# Autodesk Inventor assembly: LR_03
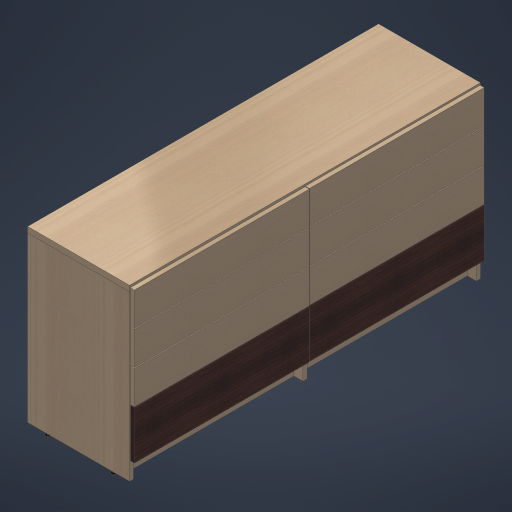
[picture p0: Inventor's stored thumbnail of the model, 512x512]
Saved by Autodesk Inventor 2024.3 (Build 283343000, 343)
## iProperties
Created: 2013-04-03
Part Number: LR_03
Document SubType Name: Assembly
Designer: User
Description: Commode
Material Code: Item.FillWorkpiece.Material.Code
Author: User
## Documents named in this file (21)
- C:\W4INV 2024 Design\PROJECTS\Living Room\Commode\LR_03.iam
- C:\W4INV 2024 Design\PROJECTS\Samples\Living Room\Commode\LR_0309.ipt
- C:\W4INV 2024 Design\PROJECTS\Samples\Living Room\Commode\LR_0304.ipt
- C:\W4INV 2024 Design\PROJECTS\Samples\Living Room\Commode\LR_0301.ipt
- C:\W4INV 2024 Design\PROJECTS\Samples\Living Room\Commode\LR_0308.ipt
- C:\W4INV 2024 Design\PROJECTS\Samples\Living Room\Commode\LR_0306.ipt
- C:\W4INV 2024 Design\PROJECTS\Samples\Living Room\Commode\LR_0303.ipt
- C:\W4INV 2024 Design\PROJECTS\Samples\Living Room\Commode\LR_0307.ipt
- C:\W4INV 2024 Design\PROJECTS\Samples\Living Room\Commode\LR_0302.ipt
- C:\W4INV 2024 Design\PROJECTS\Samples\Living Room\Commode\LR_0305.ipt
- C:\W4INV 2024 Design\PROJECTS\Samples\Living Room\Commode\SkeletonLR_030000.ipt
- C:\W4INV 2024 Design\PROJECTS\Samples\Living Room\Commode\LR_0300.ipt
- C:\W4INV 2024 Design\PROJECTS\Samples\Living Room\Commode\LR_0310.ipt
- C:\W4INV 2024 Design\PROJECTS\Samples\Living Room\Commode\LR_03\iCopy\iCopy1\LR_0311Full Pull Drawer1.iam
- C:\W4INV 2024 Design\PROJECTS\Samples\Living Room\Commode\LR_03\iCopy\iCopy2\LR_0312Full Pull Drawer1.iam
- C:\W4INV 2024 Design\_LIBRARY\Fixed joints\Minifix joint\MINIFIX D15 v2\Minifix D15 & Dowel L34 & Cap D15 PB T18 LH.ipt
- C:\W4INV 2024 Design\_LIBRARY\Fixed joints\Minifix joint\MINIFIX D15 v2\Minifix D15 & Dowel L34 & Cap D15 PB T18 RH.ipt
- C:\W4INV 2024 Design\_LIBRARY\Supports and legs\Supports\ADJUSTABLE SUPPORT\Support M6 H27 D18 with Bushing SB T18.ipt
- C:\W4INV 2024 Design\LIBRARY\Supports and legs\Supports\ADJUSTABLE SUPPORT.ipt
- C:\W4INV 2024 Design\LIBRARY\Fixed joints\Minifix joint\MINIFIX D15 v2.ipt
- C:\W4INV 2023 Design\PROJECTS\Samples\Living Room\Commode\LR_03.iam
## Components (46 placed, 17 different names)
1. K Virsus::1 — Mate:107, Mate:109, Mate:111, Mate:113, Mate:115, Mate:117
2. K Kaire::1 — Flush:4, Flush:5, Mate:55, Mate:56, Mate:57, Mate:58, Mate:59, Mate:60, Mate:63, Flush:39, Flush:69, Mate:79, Mate:81, Mate:83, Flush:72, Mate:85, Mate:87, Mate:89, Mate:91, Mate:99, Flush:83, Flush:86
3. K Desine::1 — Flush:35, Flush:71, Flush:74, Mate:97, Mate:105, Flush:85, Flush:88
4. K Vertikali pertvara::1 — Mate:61, Mate:62, Flush:37, Flush:70, Flush:73, Mate:93, Mate:95, Mate:101, Mate:103, Flush:84, Flush:87
5. K Kairys dugnas::1 — Flush:75, Flush:76, Flush:77, Flush:78, Flush:79, Flush:80, Flush:81, Flush:82
6. K Desinys dugnas::1
7. K Desine nugarele::1
8. K Kaire nugarele::1
9. K Apatinis fasadas::1 — Flush:30, Mate:54
10. K Apatinis fasadas::2 — Flush:30, Mate:54, Flush:34
11. LR_0311Full Pull Drawer1:3 [sub-assembly] — Mate:61, Flush:35, Flush:36
12. Support M6 H27 D18 with Bushing SB T18:7 — Mate:78, Flush:69, Mate:79
13. Support M6 H27 D18 with Bushing SB T18:8 — Mate:80, Flush:70, Mate:81
14. Support M6 H27 D18 with Bushing SB T18:9 — Mate:82, Flush:71, Mate:83
15. Support M6 H27 D18 with Bushing SB T18:10 — Mate:84, Flush:72, Mate:85
16. Support M6 H27 D18 with Bushing SB T18:11 — Mate:86, Flush:73, Mate:87
17. Support M6 H27 D18 with Bushing SB T18:12 — Mate:88, Flush:74, Mate:89
18. Minifix D15 & Dowel L34 & Cap D15 PB T18 LH:1 — Mate:90, Mate:91, Flush:75
19. Minifix D15 & Dowel L34 & Cap D15 PB T18 LH:2 — Mate:92, Mate:93, Flush:76
20. Minifix D15 & Dowel L34 & Cap D15 PB T18 RH:3 — Mate:94, Mate:95, Flush:77
21. Minifix D15 & Dowel L34 & Cap D15 PB T18 LH:4 — Mate:96, Mate:97, Flush:78
22. Minifix D15 & Dowel L34 & Cap D15 PB T18 LH:5 — Mate:98, Mate:99, Flush:79
23. Minifix D15 & Dowel L34 & Cap D15 PB T18 RH:6 — Mate:100, Mate:101, Flush:80
24. Minifix D15 & Dowel L34 & Cap D15 PB T18 LH:7 — Mate:102, Mate:103, Flush:81
25. Minifix D15 & Dowel L34 & Cap D15 PB T18 RH:8 — Mate:104, Mate:105, Flush:82
26. Minifix D15 & Dowel L34 & Cap D15 PB T18 LH:9 — Mate:106, Flush:83, Mate:107
27. Minifix D15 & Dowel L34 & Cap D15 PB T18 RH:10 — Mate:108, Flush:84, Mate:109
28. Minifix D15 & Dowel L34 & Cap D15 PB T18 RH:11 — Mate:110, Flush:85, Mate:111
29. Minifix D15 & Dowel L34 & Cap D15 PB T18 RH:12 — Mate:112, Flush:86, Mate:113
30. Minifix D15 & Dowel L34 & Cap D15 PB T18 LH:13 — Mate:114, Flush:87, Mate:115
31. Minifix D15 & Dowel L34 & Cap D15 PB T18 LH:14 — Mate:116, Flush:88, Mate:117
32. LR_0311Full Pull Drawer1:1 [sub-assembly] — Mate:55, Mate:56, Mate:57, Flush:36
33. LR_0312Full Pull Drawer1:1 [sub-assembly] — Mate:58, Mate:59, Mate:60, Flush:38
34. K Plintusas::1
35. K Plintusas::2
36. LR_0312Full Pull Drawer1:2 [sub-assembly] — Mate:62, Flush:37, Flush:38
37. LR_0312Full Pull Drawer1:3 [sub-assembly] — Flush:40
38. LR_0312Full Pull Drawer1:4 [sub-assembly]
39. LR_0312Full Pull Drawer1:5 [sub-assembly] — Mate:63, Flush:39, Flush:40
40. LR_0312Full Pull Drawer1:6 [sub-assembly]
41. K Virsutinis fasadas::1 — Flush:33
42. K Virsutinis fasadas::2 — Flush:33, Flush:34
43. LR_0310:3
44. LR_0310:4
45. LR_0310:5
46. LR_0310:6
## Component patterns: (2 elements, first: K Plintusas::1), (3 elements, first: LR_0312Full Pull Drawer1:2), (2 elements, first: LR_0312Full Pull Drawer1:5), (3 elements, first: K Virsutinis fasadas::1 + K Virsutinis fasadas::2)
## Relationships (83: Mate 50, Flush 33)
- Flush:4 (-80 mm): K Kaire::1
- Flush:5 (-80 mm): K Kaire::1
- Flush:12 (-16 mm)
- Flush:13 (-16 mm)
- Flush:30: K Apatinis fasadas::1 ↔ K Apatinis fasadas::2
- Mate:54 (3 mm): K Apatinis fasadas::1 ↔ K Apatinis fasadas::2
- Flush:33: K Virsutinis fasadas::1 ↔ K Virsutinis fasadas::2
- Flush:34: K Apatinis fasadas::2 ↔ K Virsutinis fasadas::2
- Mate:55: K Kaire::1 ↔ LR_0311Full Pull Drawer1:1
- Mate:56: K Kaire::1 ↔ LR_0311Full Pull Drawer1:1
- Mate:57: K Kaire::1 ↔ LR_0311Full Pull Drawer1:1
- Mate:58: K Kaire::1 ↔ LR_0312Full Pull Drawer1:1
- Mate:59: K Kaire::1 ↔ LR_0312Full Pull Drawer1:1
- Mate:60: K Kaire::1 ↔ LR_0312Full Pull Drawer1:1
- Mate:61: K Vertikali pertvara::1 ↔ LR_0311Full Pull Drawer1:3
- Flush:35: K Desine::1 ↔ LR_0311Full Pull Drawer1:3
- Flush:36: LR_0311Full Pull Drawer1:3 ↔ LR_0311Full Pull Drawer1:1
- Mate:62: K Vertikali pertvara::1 ↔ LR_0312Full Pull Drawer1:2
- Flush:37: K Vertikali pertvara::1 ↔ LR_0312Full Pull Drawer1:2
- Flush:38: LR_0312Full Pull Drawer1:1 ↔ LR_0312Full Pull Drawer1:2
- Mate:63: K Kaire::1 ↔ LR_0312Full Pull Drawer1:5
- Flush:39: K Kaire::1 ↔ LR_0312Full Pull Drawer1:5
- Flush:40: LR_0312Full Pull Drawer1:3 ↔ LR_0312Full Pull Drawer1:5
- Mate:78: Support M6 H27 D18 with Bushing SB T18:7
- Flush:69 (9 mm): K Kaire::1 ↔ Support M6 H27 D18 with Bushing SB T18:7
- Mate:79 (17.5 mm): K Kaire::1 ↔ Support M6 H27 D18 with Bushing SB T18:7
- Mate:80: Support M6 H27 D18 with Bushing SB T18:8
- Flush:70 (9 mm): K Vertikali pertvara::1 ↔ Support M6 H27 D18 with Bushing SB T18:8
- Mate:81 (17.5 mm): K Kaire::1 ↔ Support M6 H27 D18 with Bushing SB T18:8
- Mate:82: Support M6 H27 D18 with Bushing SB T18:9
- Flush:71 (9 mm): K Desine::1 ↔ Support M6 H27 D18 with Bushing SB T18:9
- Mate:83 (17.5 mm): K Kaire::1 ↔ Support M6 H27 D18 with Bushing SB T18:9
- Mate:84: Support M6 H27 D18 with Bushing SB T18:10
- Flush:72 (9 mm): K Kaire::1 ↔ Support M6 H27 D18 with Bushing SB T18:10
- Mate:85 (17.5 mm): K Kaire::1 ↔ Support M6 H27 D18 with Bushing SB T18:10
- Mate:86: Support M6 H27 D18 with Bushing SB T18:11
- Flush:73 (9 mm): K Vertikali pertvara::1 ↔ Support M6 H27 D18 with Bushing SB T18:11
- Mate:87 (17.5 mm): K Kaire::1 ↔ Support M6 H27 D18 with Bushing SB T18:11
- Mate:88: Support M6 H27 D18 with Bushing SB T18:12
- Flush:74 (9 mm): K Desine::1 ↔ Support M6 H27 D18 with Bushing SB T18:12
- Mate:89 (17.5 mm): K Kaire::1 ↔ Support M6 H27 D18 with Bushing SB T18:12
- Mate:90: Minifix D15 & Dowel L34 & Cap D15 PB T18 LH:1
- Mate:91: K Kaire::1 ↔ Minifix D15 & Dowel L34 & Cap D15 PB T18 LH:1
- Flush:75 (18 mm): K Kairys dugnas::1 ↔ Minifix D15 & Dowel L34 & Cap D15 PB T18 LH:1
- Mate:92: Minifix D15 & Dowel L34 & Cap D15 PB T18 LH:2
- Mate:93: K Vertikali pertvara::1 ↔ Minifix D15 & Dowel L34 & Cap D15 PB T18 LH:2
- Flush:76 (18 mm): K Kairys dugnas::1 ↔ Minifix D15 & Dowel L34 & Cap D15 PB T18 LH:2
- Mate:94: Minifix D15 & Dowel L34 & Cap D15 PB T18 RH:3
- Mate:95: K Vertikali pertvara::1 ↔ Minifix D15 & Dowel L34 & Cap D15 PB T18 RH:3
- Flush:77 (18 mm): K Kairys dugnas::1 ↔ Minifix D15 & Dowel L34 & Cap D15 PB T18 RH:3
- Mate:96: Minifix D15 & Dowel L34 & Cap D15 PB T18 LH:4
- Mate:97: K Desine::1 ↔ Minifix D15 & Dowel L34 & Cap D15 PB T18 LH:4
- Flush:78 (18 mm): K Kairys dugnas::1 ↔ Minifix D15 & Dowel L34 & Cap D15 PB T18 LH:4
- Mate:98: Minifix D15 & Dowel L34 & Cap D15 PB T18 LH:5
- Mate:99: K Kaire::1 ↔ Minifix D15 & Dowel L34 & Cap D15 PB T18 LH:5
- Flush:79 (18 mm): K Kairys dugnas::1 ↔ Minifix D15 & Dowel L34 & Cap D15 PB T18 LH:5
- Mate:100: Minifix D15 & Dowel L34 & Cap D15 PB T18 RH:6
- Mate:101: K Vertikali pertvara::1 ↔ Minifix D15 & Dowel L34 & Cap D15 PB T18 RH:6
- Flush:80 (18 mm): K Kairys dugnas::1 ↔ Minifix D15 & Dowel L34 & Cap D15 PB T18 RH:6
- Mate:102: Minifix D15 & Dowel L34 & Cap D15 PB T18 LH:7
- Mate:103: K Vertikali pertvara::1 ↔ Minifix D15 & Dowel L34 & Cap D15 PB T18 LH:7
- Flush:81 (18 mm): K Kairys dugnas::1 ↔ Minifix D15 & Dowel L34 & Cap D15 PB T18 LH:7
- Mate:104: Minifix D15 & Dowel L34 & Cap D15 PB T18 RH:8
- Mate:105: K Desine::1 ↔ Minifix D15 & Dowel L34 & Cap D15 PB T18 RH:8
- Flush:82 (18 mm): K Kairys dugnas::1 ↔ Minifix D15 & Dowel L34 & Cap D15 PB T18 RH:8
- Mate:106: Minifix D15 & Dowel L34 & Cap D15 PB T18 LH:9
- Flush:83 (18 mm): K Kaire::1 ↔ Minifix D15 & Dowel L34 & Cap D15 PB T18 LH:9
- Mate:107: K Virsus::1 ↔ Minifix D15 & Dowel L34 & Cap D15 PB T18 LH:9
- Mate:108: Minifix D15 & Dowel L34 & Cap D15 PB T18 RH:10
- Flush:84 (18 mm): K Vertikali pertvara::1 ↔ Minifix D15 & Dowel L34 & Cap D15 PB T18 RH:10
- Mate:109: K Virsus::1 ↔ Minifix D15 & Dowel L34 & Cap D15 PB T18 RH:10
- Mate:110: Minifix D15 & Dowel L34 & Cap D15 PB T18 RH:11
- Flush:85 (18 mm): K Desine::1 ↔ Minifix D15 & Dowel L34 & Cap D15 PB T18 RH:11
- Mate:111: K Virsus::1 ↔ Minifix D15 & Dowel L34 & Cap D15 PB T18 RH:11
- Mate:112: Minifix D15 & Dowel L34 & Cap D15 PB T18 RH:12
- Flush:86 (18 mm): K Kaire::1 ↔ Minifix D15 & Dowel L34 & Cap D15 PB T18 RH:12
- Mate:113: K Virsus::1 ↔ Minifix D15 & Dowel L34 & Cap D15 PB T18 RH:12
- Mate:114: Minifix D15 & Dowel L34 & Cap D15 PB T18 LH:13
- Flush:87 (18 mm): K Vertikali pertvara::1 ↔ Minifix D15 & Dowel L34 & Cap D15 PB T18 LH:13
- Mate:115: K Virsus::1 ↔ Minifix D15 & Dowel L34 & Cap D15 PB T18 LH:13
- Mate:116: Minifix D15 & Dowel L34 & Cap D15 PB T18 LH:14
- Flush:88 (18 mm): K Desine::1 ↔ Minifix D15 & Dowel L34 & Cap D15 PB T18 LH:14
- Mate:117: K Virsus::1 ↔ Minifix D15 & Dowel L34 & Cap D15 PB T18 LH:14
